# Autodesk Inventor assembly: 3_8 Shawny Lift 40t Idler
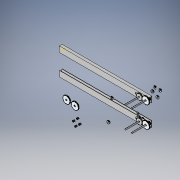
[picture p0: Inventor's stored thumbnail of the model, 180x180]
Saved by Autodesk Inventor 2018 (Build 220112000, 112)
## iProperties
Created: 2019-01-14
Part Number: 3_8 Shawny Lift 40t Idler
Document SubType Name: Assembly
Designer: Gabriel
Author: Gabriel
## Documents named in this file (9)
- C:\Users\Gabriel\Documents\3_8 Shawny Lift 40t Idler.iam
- C:\Users\Gabriel\Documents\8T spur gear 775.ipt
- C:\Users\Gabriel\Documents\36in Aluminum Channel.ipt
- C:\Users\Gabriel\Documents\Sanded Hex Rod.ipt
- C:\Users\Gabriel\Documents\Spacer 1 16 in.ipt
- C:\Users\Gabriel\Documents\Flanged bearing 3 8 in .ipt
- C:\Users\Gabriel\Documents\am-2300 Collar Clamp, 0.375'' Hex Bore, Aluminum REV2.iam
- C:\Users\Gabriel\Documents\50t 20dp 3 8 in gear.ipt
- C:\Users\Gabriel\Documents\40t_Aluminum_Spur_Gear_20_DP_3_8_Hex_Bore_217-2707.ipt
## Components (36 placed, 8 different names)
1. 8T spur gear 775:1
2. 8T spur gear 775:2
3. 8T spur gear 775:3
4. 8T spur gear 775:4
5. 36in Aluminum Channel:1 — Mate:1, Mate:2, Mate:3, Mate:4, Mate:5, Mate:6, Mate:7, Mate:8
6. Sanded Hex Rod:1 — Mate:25, Mate:26, Mate:29, Mate:30, Mate:35, Mate:36
7. 36in Aluminum Channel:2 — Mate:13, Mate:14, Mate:15, Mate:16, Mate:17, Mate:18, Mate:19, Mate:20
8. Sanded Hex Rod:4 — Mate:41, Mate:42, Mate:45, Mate:46, Mate:51, Mate:52
9. Flanged bearing 3 8 in :1 — Mate:13, Mate:14, Mate:31
10. Flanged bearing 3 8 in :2 — Mate:3, Mate:4, Mate:41, Mate:42
11. Flanged bearing 3 8 in :6 — Mate:1, Mate:2, Mate:47
12. Flanged bearing 3 8 in :7 — Mate:15, Mate:16, Mate:25, Mate:26
13. am-2300 Collar Clamp, 0.375'' Hex Bore, Aluminum REV2:1 [sub-assembly]
14. am-2300 Collar Clamp, 0.375'' Hex Bore, Aluminum REV2:2 [sub-assembly]
15. am-2300 Collar Clamp, 0.375'' Hex Bore, Aluminum REV2:3 [sub-assembly]
16. am-2300 Collar Clamp, 0.375'' Hex Bore, Aluminum REV2:5 [sub-assembly]
17. am-2300 Collar Clamp, 0.375'' Hex Bore, Aluminum REV2:7 [sub-assembly]
18. am-2300 Collar Clamp, 0.375'' Hex Bore, Aluminum REV2:8 [sub-assembly]
19. Spacer 1 16 in:3
20. Spacer 1 16 in:4
21. Spacer 1 16 in:5 — Mate:29, Mate:30, Mate:31, Mate:37
22. Spacer 1 16 in:6 — Mate:48, Mate:49, Mate:50, Mate:56
23. Spacer 1 16 in:7 — Mate:32, Mate:33, Mate:34, Mate:40
24. Spacer 1 16 in:8 — Mate:45, Mate:46, Mate:47, Mate:53
25. 50t 20dp 3 8 in gear:1 — Mate:35, Mate:36, Mate:37
26. 50t 20dp 3 8 in gear:4 — Mate:51, Mate:52, Mate:53
27. 50t 20dp 3 8 in gear:5
28. 50t 20dp 3 8 in gear:7
29. Flanged bearing 3 8 in :8 — Mate:19, Mate:20, Mate:27, Mate:28
30. Flanged bearing 3 8 in :11 — Mate:7, Mate:8, Mate:43, Mate:44
31. Flanged bearing 3 8 in :13 — Mate:17, Mate:18, Mate:34
32. Flanged bearing 3 8 in :15 — Mate:5, Mate:6, Mate:50
33. Sanded Hex Rod:5 — Mate:43, Mate:44, Mate:48, Mate:49, Mate:54, Mate:55
34. Sanded Hex Rod:8 — Mate:27, Mate:28, Mate:32, Mate:33, Mate:38, Mate:39
35. 40t_Aluminum_Spur_Gear_20_DP_3_8_Hex_Bore_217-2707:1 — Mate:38, Mate:39, Mate:40
36. 40t_Aluminum_Spur_Gear_20_DP_3_8_Hex_Bore_217-2707:2 — Mate:54, Mate:55, Mate:56
## Relationships (48: Mate 48)
- Mate:1: 36in Aluminum Channel:1 ↔ Flanged bearing 3 8 in :6
- Mate:2: 36in Aluminum Channel:1 ↔ Flanged bearing 3 8 in :6
- Mate:3: 36in Aluminum Channel:1 ↔ Flanged bearing 3 8 in :2
- Mate:4: 36in Aluminum Channel:1 ↔ Flanged bearing 3 8 in :2
- Mate:5: 36in Aluminum Channel:1 ↔ Flanged bearing 3 8 in :15
- Mate:6: 36in Aluminum Channel:1 ↔ Flanged bearing 3 8 in :15
- Mate:7: 36in Aluminum Channel:1 ↔ Flanged bearing 3 8 in :11
- Mate:8: 36in Aluminum Channel:1 ↔ Flanged bearing 3 8 in :11
- Mate:13: 36in Aluminum Channel:2 ↔ Flanged bearing 3 8 in :1
- Mate:14: 36in Aluminum Channel:2 ↔ Flanged bearing 3 8 in :1
- Mate:15: 36in Aluminum Channel:2 ↔ Flanged bearing 3 8 in :7
- Mate:16: 36in Aluminum Channel:2 ↔ Flanged bearing 3 8 in :7
- Mate:17: 36in Aluminum Channel:2 ↔ Flanged bearing 3 8 in :13
- Mate:18: 36in Aluminum Channel:2 ↔ Flanged bearing 3 8 in :13
- Mate:19: 36in Aluminum Channel:2 ↔ Flanged bearing 3 8 in :8
- Mate:20: 36in Aluminum Channel:2 ↔ Flanged bearing 3 8 in :8
- Mate:25: Sanded Hex Rod:1 ↔ Flanged bearing 3 8 in :7
- Mate:26: Sanded Hex Rod:1 ↔ Flanged bearing 3 8 in :7
- Mate:27: Flanged bearing 3 8 in :8 ↔ Sanded Hex Rod:8
- Mate:28: Flanged bearing 3 8 in :8 ↔ Sanded Hex Rod:8
- Mate:29: Sanded Hex Rod:1 ↔ Spacer 1 16 in:5
- Mate:30: Sanded Hex Rod:1 ↔ Spacer 1 16 in:5
- Mate:31: Flanged bearing 3 8 in :1 ↔ Spacer 1 16 in:5
- Mate:32: Spacer 1 16 in:7 ↔ Sanded Hex Rod:8
- Mate:33: Spacer 1 16 in:7 ↔ Sanded Hex Rod:8
- Mate:34: Spacer 1 16 in:7 ↔ Flanged bearing 3 8 in :13
- Mate:35: Sanded Hex Rod:1 ↔ 50t 20dp 3 8 in gear:1
- Mate:36: Sanded Hex Rod:1 ↔ 50t 20dp 3 8 in gear:1
- Mate:37: Spacer 1 16 in:5 ↔ 50t 20dp 3 8 in gear:1
- Mate:38: Sanded Hex Rod:8 ↔ 40t_Aluminum_Spur_Gear_20_DP_3_8_Hex_Bore_217-2707:1
- Mate:39: Sanded Hex Rod:8 ↔ 40t_Aluminum_Spur_Gear_20_DP_3_8_Hex_Bore_217-2707:1
- Mate:40: Spacer 1 16 in:7 ↔ 40t_Aluminum_Spur_Gear_20_DP_3_8_Hex_Bore_217-2707:1
- Mate:41: Sanded Hex Rod:4 ↔ Flanged bearing 3 8 in :2
- Mate:42: Sanded Hex Rod:4 ↔ Flanged bearing 3 8 in :2
- Mate:43: Flanged bearing 3 8 in :11 ↔ Sanded Hex Rod:5
- Mate:44: Flanged bearing 3 8 in :11 ↔ Sanded Hex Rod:5
- Mate:45: Sanded Hex Rod:4 ↔ Spacer 1 16 in:8
- Mate:46: Sanded Hex Rod:4 ↔ Spacer 1 16 in:8
- Mate:47: Flanged bearing 3 8 in :6 ↔ Spacer 1 16 in:8
- Mate:48: Spacer 1 16 in:6 ↔ Sanded Hex Rod:5
- Mate:49: Spacer 1 16 in:6 ↔ Sanded Hex Rod:5
- Mate:50: Spacer 1 16 in:6 ↔ Flanged bearing 3 8 in :15
- Mate:51: Sanded Hex Rod:4 ↔ 50t 20dp 3 8 in gear:4
- Mate:52: Sanded Hex Rod:4 ↔ 50t 20dp 3 8 in gear:4
- Mate:53: Spacer 1 16 in:8 ↔ 50t 20dp 3 8 in gear:4
- Mate:54: Sanded Hex Rod:5 ↔ 40t_Aluminum_Spur_Gear_20_DP_3_8_Hex_Bore_217-2707:2
- Mate:55: Sanded Hex Rod:5 ↔ 40t_Aluminum_Spur_Gear_20_DP_3_8_Hex_Bore_217-2707:2
- Mate:56: Spacer 1 16 in:6 ↔ 40t_Aluminum_Spur_Gear_20_DP_3_8_Hex_Bore_217-2707:2
